# Autodesk Inventor assembly: Mash Tank Box
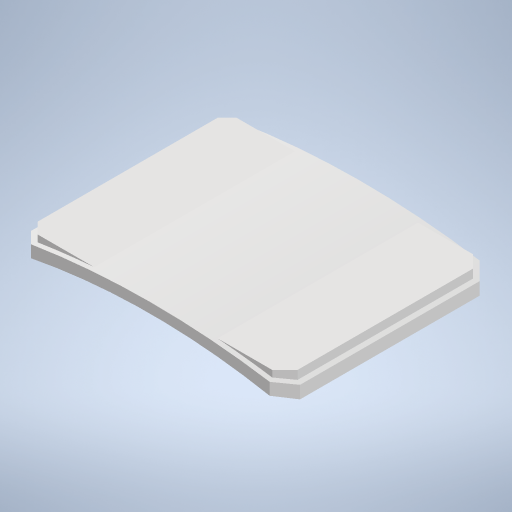
[picture p0: Inventor's stored thumbnail of the model, 512x512]
Saved by Autodesk Inventor 2024 (Build 280153000, 153)
## iProperties
Created: 2024-12-24
Part Number: Mash Tank Box
Document SubType Name: Assembly
Designer: Emil
Author: Emil
## Documents named in this file (3)
- C:\Users\Emil\OneDrive\Dokument\Projekt-Emil\MachMachine\InventorCad\Mash tank box\Mash Tank Box.iam
- C:\Users\Emil\OneDrive\Dokument\Projekt-Emil\MachMachine\InventorCad\Mash tank box\Solid8.ipt
- C:\Users\Emil\OneDrive\Dokument\Projekt-Emil\MachMachine\InventorCad\Mash tank box\Solid9.ipt
## Components (2 placed, 2 different names)
1. Solid8:1 — Rigid:1
2. Solid9:1 — Rigid:1
## Relationships (1: WeldJoint 1)
- Rigid:1 [WeldJoint]: Solid8:1 ↔ Solid9:1
